# Autodesk Inventor assembly: RealSense100
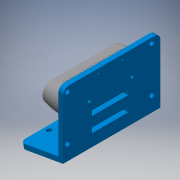
[picture p0: Inventor's stored thumbnail of the model, 180x180]
Saved by Autodesk Inventor 2019 (Build 230136000, 136)
## iProperties
Created: 2019-12-23
Part Number: RealSense100
Document SubType Name: Assembly
Designer: james
Author: james
## Documents named in this file (3)
- F:\JimsRobot\FIRSTRobots\Design\Library\Jims\RealSense100.iam
- F:\JimsRobot\FIRSTRobots\Design\Library\Jims\Realsense100.ipt
- F:\JimsRobot\FIRSTRobots\Design\Library\Intel\Intel_RealSense_Depth_Camera_D435.iam
## Components (2 placed, 2 different names)
1. Realsense100:1 — Mate:1, Mate:2, Mate:3
2. Intel_RealSense_Depth_Camera_D435:1 [sub-assembly] — Mate:1, Mate:2, Mate:3
## Relationships (3: Mate 3)
- Mate:1: Realsense100:1 ↔ Intel_RealSense_Depth_Camera_D435:1
- Mate:2: Realsense100:1 ↔ Intel_RealSense_Depth_Camera_D435:1
- Mate:3: Realsense100:1 ↔ Intel_RealSense_Depth_Camera_D435:1
